# Autodesk Inventor assembly: Base 02
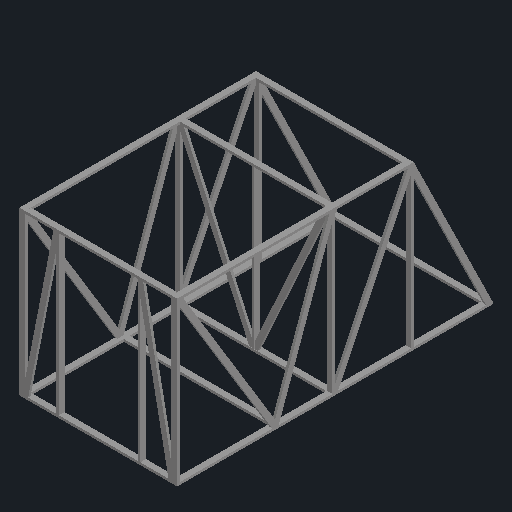
[picture p0: Inventor's stored thumbnail of the model, 512x512]
Saved by Autodesk Inventor 2026 (Build 300175000, 175)
## iProperties
Created: 2024-09-16
Part Number: Base 02
Document SubType Name: Assembly
Designer: User
Author: User
## Documents named in this file (10)
- C:\Users\trott\Documents\UofSC-ASME-Tiger-Burn-Design-2025\CAD\Body\Base 02\Base 02.iam
- C:\Users\trott\Documents\UofSC-ASME-Tiger-Burn-Design-2025\CAD\Body\Base 02\16'x2x4.ipt
- C:\Users\trott\Documents\UofSC-ASME-Tiger-Burn-Design-2025\CAD\Body\Base 02\7'5x2x4.ipt
- C:\Users\trott\Documents\UofSC-ASME-Tiger-Burn-Design-2025\CAD\Body\Base 02\10'x2x4.ipt
- C:\Users\trott\Documents\UofSC-ASME-Tiger-Burn-Design-2025\CAD\Body\Base 02\12'x2x4.ipt
- C:\Users\trott\Documents\UofSC-ASME-Tiger-Burn-Design-2025\CAD\Body\Base 02\s48'x2x4.ipt
- C:\Users\trott\Documents\UofSC-ASME-Tiger-Burn-Design-2025\CAD\Body\Base 02\s48x2x4b.ipt
- C:\Users\trott\Documents\UofSC-ASME-Tiger-Burn-Design-2025\CAD\Body\Base 02\s58x2x4.ipt
- C:\Users\trott\Documents\UofSC-ASME-Tiger-Burn-Design-2025\CAD\Body\Base 02\s28x2x4.ipt
- C:\Users\trott\Documents\UofSC-ASME-Tiger-Burn-Design-2025\CAD\Body\Base 02\side1.ipt
## Components (30 placed, 9 different names)
1. 16'x2x4:1 — Flush:1, Mate:1, Flush:2, Flush:14, Mate:8, Flush:15, Mate:9, Flush:16, Flush:19, Mate:12, Flush:22, Mate:23, Flush:37, Mate:28, Flush:44
2. 16'x2x4:2 — Flush:1, Mate:1, Flush:2, Flush:3, Mate:2, Flush:4, Flush:5, Flush:6, Flush:8, Flush:9, Mate:3, Mate:5, Mate:6, Flush:12, Mate:7, Flush:13, Flush:17, Mate:10, Mate:11, Flush:18, Flush:23, Mate:20, Flush:43
3. 7'5x2x4:1 — Flush:3, Mate:2, Flush:4, Flush:10, Flush:34, Flush:35
4. 7'5x2x4:2 — Flush:5, Mate:6, Flush:10
5. 7'5x2x4:3 — Flush:6, Mate:5, Flush:11, Flush:20, Flush:21, Flush:31, Flush:38, Mate:24
6. 7'5x2x4:5 — Flush:8, Flush:9, Mate:3, Flush:11
7. 10'x2x4:1 — Flush:12, Mate:7, Flush:13, Flush:24, Flush:25, Flush:33
8. 10'x2x4:2 — Flush:14, Mate:8, Flush:15, Mate:14, Flush:26, Flush:27, Flush:45
9. 10'x2x4:3 — Mate:9, Flush:16, Flush:21, Flush:39, Flush:42, Mate:27
10. 10'x2x4:4 — Flush:17, Mate:10, Flush:20, Mate:25, Flush:41, Flush:47
11. 10'x2x4:5 — Flush:19, Mate:12, Flush:22, Mate:22, Mate:31, Flush:48
12. 10'x2x4:6 — Mate:11, Flush:18, Flush:23, Mate:13, Flush:28, Flush:36
13. 12'x2x4:1 — Mate:13, Flush:24, Flush:25, Mate:16, Flush:32
14. 12'x2x4:2 — Mate:14, Flush:26, Flush:27, Mate:15, Flush:29, Flush:30, Mate:17, Mate:32
15. 7'5x2x4:6 — Flush:28, Mate:15, Flush:29
16. 7'5x2x4:7 — Flush:30, Flush:31, Mate:16, Mate:26
17. 7'5x2x4:8 — Flush:32, Flush:33, Mate:17, Mate:18, Mate:19, Mate:30
18. 10'x2x4:7 — Flush:35, Mate:19, Mate:20, Mate:21, Mate:29, Flush:46
19. 10'x2x4:8 — Flush:34, Mate:18, Mate:21
20. s48'x2x4:1 — Flush:36
21. s48'x2x4:2 — Mate:22, Mate:23, Flush:37
22. 10'x2x4:9 — Flush:38, Mate:24, Flush:39
23. s48x2x4b:1 — Flush:42
24. s48x2x4b:2 — Mate:25, Mate:26, Flush:41
25. s58x2x4:1 — Flush:43
26. s58x2x4:2 — Mate:27, Mate:28, Flush:44
27. s28x2x4:1 — Flush:45
28. s28x2x4:2 — Mate:29, Mate:30, Flush:46
29. side1:1 — Flush:47
30. side1:2 — Mate:31, Mate:32, Flush:48
## Relationships (77: Flush 46, Mate 31)
- Flush:1: 16'x2x4:1 ↔ 16'x2x4:2
- Mate:1 (-2438.4 mm): 16'x2x4:1 ↔ 16'x2x4:2
- Flush:2: 16'x2x4:1 ↔ 16'x2x4:2
- Flush:3: 16'x2x4:2 ↔ 7'5x2x4:1
- Mate:2: 16'x2x4:2 ↔ 7'5x2x4:1
- Flush:4: 16'x2x4:2 ↔ 7'5x2x4:1
- Flush:5: 16'x2x4:2 ↔ 7'5x2x4:2
- Flush:6: 16'x2x4:2 ↔ 7'5x2x4:3
- Flush:8: 16'x2x4:2 ↔ 7'5x2x4:5
- Flush:9: 16'x2x4:2 ↔ 7'5x2x4:5
- Mate:3: 16'x2x4:2 ↔ 7'5x2x4:5
- Mate:5: 16'x2x4:2 ↔ 7'5x2x4:3
- Mate:6: 16'x2x4:2 ↔ 7'5x2x4:2
- Flush:10 (-1524 mm): 7'5x2x4:1 ↔ 7'5x2x4:2
- Flush:11 (-2393.95 mm): 7'5x2x4:3 ↔ 7'5x2x4:5
- Flush:12: 16'x2x4:2 ↔ 10'x2x4:1
- Mate:7: 16'x2x4:2 ↔ 10'x2x4:1
- Flush:13: 16'x2x4:2 ↔ 10'x2x4:1
- Flush:14: 16'x2x4:1 ↔ 10'x2x4:2
- Mate:8: 16'x2x4:1 ↔ 10'x2x4:2
- Flush:15: 16'x2x4:1 ↔ 10'x2x4:2
- Mate:9: 16'x2x4:1 ↔ 10'x2x4:3
- Flush:16: 16'x2x4:1 ↔ 10'x2x4:3
- Flush:17: 16'x2x4:2 ↔ 10'x2x4:4
- Mate:10: 16'x2x4:2 ↔ 10'x2x4:4
- Mate:11: 16'x2x4:2 ↔ 10'x2x4:6
- Flush:18: 16'x2x4:2 ↔ 10'x2x4:6
- Flush:19: 16'x2x4:1 ↔ 10'x2x4:5
- Mate:12: 16'x2x4:1 ↔ 10'x2x4:5
- Flush:20 (44.45 mm): 7'5x2x4:3 ↔ 10'x2x4:4
- Flush:21 (-44.45 mm): 7'5x2x4:3 ↔ 10'x2x4:3
- Flush:22 (-1219.2 mm): 16'x2x4:1 ↔ 10'x2x4:5
- Flush:23 (1219.2 mm): 16'x2x4:2 ↔ 10'x2x4:6
- Mate:13: 10'x2x4:6 ↔ 12'x2x4:1
- Flush:24: 10'x2x4:1 ↔ 12'x2x4:1
- Flush:25: 10'x2x4:1 ↔ 12'x2x4:1
- Mate:14: 10'x2x4:2 ↔ 12'x2x4:2
- Flush:26: 10'x2x4:2 ↔ 12'x2x4:2
- Flush:27: 10'x2x4:2 ↔ 12'x2x4:2
- Flush:28: 10'x2x4:6 ↔ 7'5x2x4:6
- Mate:15: 12'x2x4:2 ↔ 7'5x2x4:6
- Flush:29: 12'x2x4:2 ↔ 7'5x2x4:6
- Flush:30: 12'x2x4:2 ↔ 7'5x2x4:7
- Flush:31: 7'5x2x4:3 ↔ 7'5x2x4:7
- Mate:16: 12'x2x4:1 ↔ 7'5x2x4:7
- Flush:32: 12'x2x4:1 ↔ 7'5x2x4:8
- Flush:33: 10'x2x4:1 ↔ 7'5x2x4:8
- Mate:17: 12'x2x4:2 ↔ 7'5x2x4:8
- Flush:34: 7'5x2x4:1 ↔ 10'x2x4:8
- Mate:18: 7'5x2x4:8 ↔ 10'x2x4:8
- Flush:35: 7'5x2x4:1 ↔ 10'x2x4:7
- Mate:19: 7'5x2x4:8 ↔ 10'x2x4:7
- Mate:20 (-609.6 mm): 16'x2x4:2 ↔ 10'x2x4:7
- Mate:21 (1219.2 mm): 10'x2x4:7 ↔ 10'x2x4:8
- Flush:36: 10'x2x4:6 ↔ s48'x2x4:1
- Mate:22: 10'x2x4:5 ↔ s48'x2x4:2
- Mate:23: 16'x2x4:1 ↔ s48'x2x4:2
- Flush:37: 16'x2x4:1 ↔ s48'x2x4:2
- Flush:38: 7'5x2x4:3 ↔ 10'x2x4:9
- Mate:24: 7'5x2x4:3 ↔ 10'x2x4:9
- Flush:39 (1200.15 mm): 10'x2x4:3 ↔ 10'x2x4:9
- Mate:25: 10'x2x4:4 ↔ s48x2x4b:2
- Mate:26: 7'5x2x4:7 ↔ s48x2x4b:2
- Flush:41: 10'x2x4:4 ↔ s48x2x4b:2
- Flush:42: 10'x2x4:3 ↔ s48x2x4b:1
- Flush:43: 16'x2x4:2 ↔ s58x2x4:1
- Mate:27: 10'x2x4:3 ↔ s58x2x4:2
- Mate:28: 16'x2x4:1 ↔ s58x2x4:2
- Flush:44: 16'x2x4:1 ↔ s58x2x4:2
- Flush:45: 10'x2x4:2 ↔ s28x2x4:1
- Mate:29: 10'x2x4:7 ↔ s28x2x4:2
- Mate:30: 7'5x2x4:8 ↔ s28x2x4:2
- Flush:46: 10'x2x4:7 ↔ s28x2x4:2
- Flush:47: 10'x2x4:4 ↔ side1:1
- Mate:31: 10'x2x4:5 ↔ side1:2
- Mate:32: 12'x2x4:2 ↔ side1:2
- Flush:48: 10'x2x4:5 ↔ side1:2
